# Autodesk Inventor assembly: fuse
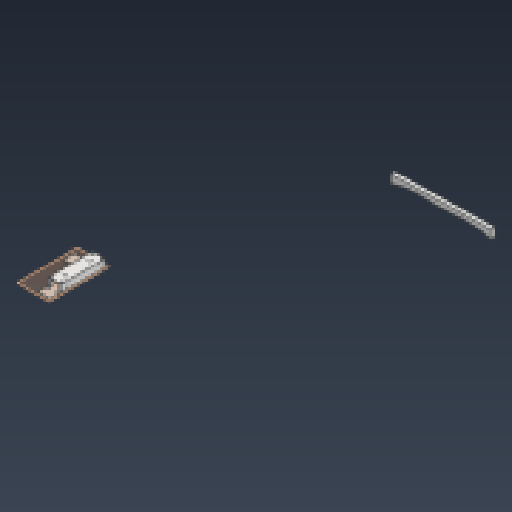
[picture p0: Inventor's stored thumbnail of the model, 512x512]
Saved by Autodesk Inventor 2023 (Build 270158000, 158)
## iProperties
Created: 2025-12-26
Part Number: fuse
Document SubType Name: Assembly
Designer: szymo
Author: szymo
## Documents named in this file (4)
- D:\tech\diy\e-skateboard\projekcik-inventor\steps\fuse.iam
- D:\tech\diy\e-skateboard\projekcik-inventor\other-parts\steps\fusion_hold.ipt
- D:\tech\diy\e-skateboard\projekcik-inventor\other-parts\deseczka_dol_check - 7.ipt
- D:\tech\diy\e-skateboard\projekcik-inventor\steps\fuse_holder_cover.ipt
## Components (3 placed, 3 different names)
1. fuse_holder_cover:1
2. deseczka_dol_check - 7:1
3. fusion_hold:1
## Relationships (2: Flush 2)
- [Flush]: fuse_holder_cover:1 ↔ fusion_hold:1
- [Flush]: fuse_holder_cover:1 ↔ fusion_hold:1
